# Autodesk Inventor assembly: Dock_OBC_TRX
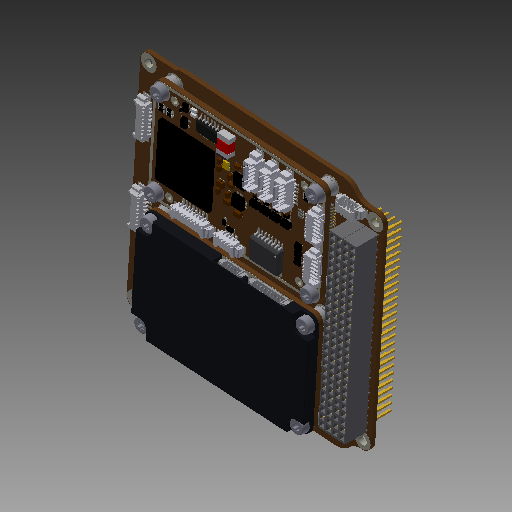
[picture p0: Inventor's stored thumbnail of the model, 512x512]
Saved by Autodesk Inventor 2017 (Build 210142000, 142)
## iProperties
Created: 2016-03-16
Part Number: Dock_OBC_TRX
Document SubType Name: Assembly
Designer: Cosmonauta
Author: Cosmonauta
## Documents named in this file (4)
- C:\Users\Cosmonauta\ownCloud\Aurora\Proyectos\SUCHAI_2-3\Subsistemas\MEC\CAD_Cubesat3U\NanoDock_OBC_TRX\Dock_OBC_TRX.iam
- C:\Users\Cosmonauta\ownCloud\Aurora\Proyectos\SUCHAI_2-3\Subsistemas\MEC\CAD_Cubesat3U\NanoDock\CAD\Motherboard.iam
- C:\Users\Cosmonauta\ownCloud\Aurora\Proyectos\SUCHAI_2-3\Subsistemas\MEC\CAD_Cubesat3U\Nanocom_AX100\CAD\ax100-2.iam
- C:\Users\Cosmonauta\ownCloud\Aurora\Proyectos\SUCHAI_2-3\Subsistemas\MEC\CAD_Cubesat3U\Nanomind_A3200\CAD\nanomind-a3200-3.iam
## Components (3 placed, 3 different names)
1. Motherboard:1 [sub-assembly] — Mate:1, Mate:2, Mate:3, Mate:4, Mate:5, Mate:6
2. ax100-2:1 [sub-assembly] — Mate:1, Mate:2, Mate:3
3. nanomind-a3200-3:1 [sub-assembly] — Mate:4, Mate:5, Mate:6
## Relationships (6: Mate 6)
- Mate:1: Motherboard:1 ↔ ax100-2:1
- Mate:2: Motherboard:1 ↔ ax100-2:1
- Mate:3: Motherboard:1 ↔ ax100-2:1
- Mate:4: Motherboard:1 ↔ nanomind-a3200-3:1
- Mate:5: Motherboard:1 ↔ nanomind-a3200-3:1
- Mate:6: Motherboard:1 ↔ nanomind-a3200-3:1
